# Autodesk Inventor assembly: TAZ 6 Gantry Convex Model
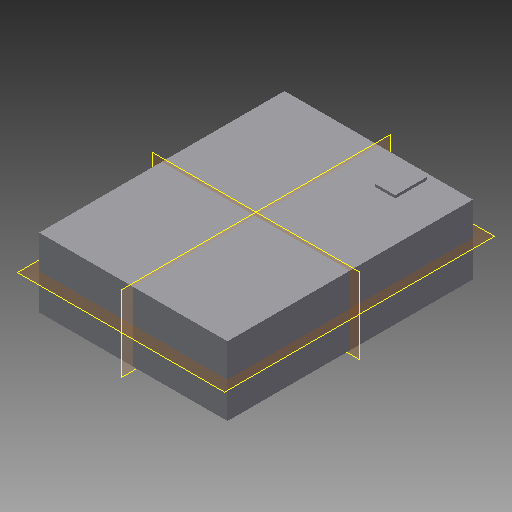
[picture p0: Inventor's stored thumbnail of the model, 512x512]
Saved by Autodesk Inventor 2019 (Build 230136000, 136)
## iProperties
Created: 2021-05-14
Part Number: TAZ 6 Gantry Convex Model
Document SubType Name: Assembly
Designer: Eric
Author: Eric
## Documents named in this file (3)
- C:\Users\Eric\Documents\! - Uni\Year 4\MENG-Robot-Fab-Project\Models\For_Optimiser\Static Parts Assembly\TAZ 6 Assembly\TAZ 6 Gantry Convex Model.iam
- C:\Users\Eric\Documents\! - Uni\Year 4\MENG-Robot-Fab-Project\Models\For_Optimiser\Static Parts Assembly\TAZ 6 Assembly\TAZ6Gantry_1.ipt
- C:\Users\Eric\Documents\! - Uni\Year 4\MENG-Robot-Fab-Project\Models\For_Optimiser\Static Parts Assembly\TAZ 6 Assembly\TAZ6Gantry_2.ipt
## Components (2 placed, 2 different names)
1. TAZ6Gantry_1:1 — Symmetry:1
2. TAZ6Gantry_2:1 — Symmetry:1
## Relationships (1: Symmetry 1)
- Symmetry:1: TAZ6Gantry_1:1 ↔ TAZ6Gantry_2:1
